# Autodesk Inventor assembly: SunTracerAssembly
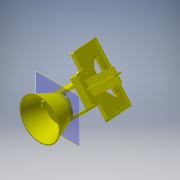
[picture p0: Inventor's stored thumbnail of the model, 180x180]
Saved by Autodesk Inventor 2017 (Build 210142000, 142)
## iProperties
Created: 2019-02-02
Part Number: SunTracerAssembly
Document SubType Name: Assembly
Designer: Denis Kurka
Author: Denis Kurka
## Documents named in this file (6)
- C:\Users\Denis Kurka\Desktop\NAG\Meteostanice\SunTracer\SunTracerAssembly.iam
- C:\Users\Denis Kurka\Desktop\NAG\Meteostanice\SunTracer\zaklad.ipt
- C:\Users\Denis Kurka\Desktop\NAG\Meteostanice\SunTracer\hlava.ipt
- C:\Users\Denis Kurka\Desktop\NAG\Meteostanice\SunTracer\rameno.ipt
- C:\Users\Denis Kurka\Desktop\NAG\Meteostanice\SunTracer\drzaksolaru.ipt
- C:\Users\Denis Kurka\Desktop\NAG\Meteostanice\SunTracer\drzakfotorezistoru.ipt
## Components (5 placed, 5 different names)
1. zaklad:1 — Mate:1, Mate:2
2. hlava:1 — Mate:1, Mate:2, Mate:3, Mate:4
3. rameno:1 — Mate:3, Mate:4, Mate:5, Flush:1, Flush:2
4. drzaksolaru:1 — Mate:5, Flush:1, Flush:2, Mate:6, Flush:3, Flush:4
5. drzakfotorezistoru:1 — Mate:6, Flush:3, Flush:4
## Relationships (10: Mate 6, Flush 4)
- Mate:1: zaklad:1 ↔ hlava:1
- Mate:2: zaklad:1 ↔ hlava:1
- Mate:3: hlava:1 ↔ rameno:1
- Mate:4: hlava:1 ↔ rameno:1
- Mate:5: rameno:1 ↔ drzaksolaru:1
- Flush:1 (-35 mm): rameno:1 ↔ drzaksolaru:1
- Flush:2 (12 mm): rameno:1 ↔ drzaksolaru:1
- Mate:6: drzaksolaru:1 ↔ drzakfotorezistoru:1
- Flush:3: drzaksolaru:1 ↔ drzakfotorezistoru:1
- Flush:4: drzaksolaru:1 ↔ drzakfotorezistoru:1
